# Autodesk Inventor assembly: switchplate-2
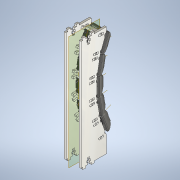
[picture p0: Inventor's stored thumbnail of the model, 180x180]
Saved by Autodesk Inventor 2020.1 (Build 241239000, 239)
## iProperties
Created: 2019-07-06
Part Number: switchplate-2
Document SubType Name: Assembly
Designer: Thibault
Mass: 36.7321 g
Surface Area: 336.688 cm^2
Volume: 13.7102 cm^3
Density: 2.67918 g/cm^3
Author: Thibault
## Documents named in this file (7)
- C:\Users\Thibault Polge\Documents\Habilis\mech\switchplate\switchplate-2.iam
- C:\Users\Thibault Polge\Documents\Habilis\mech\switchplate_support.ipt
- C:\Users\Thibault Polge\Documents\Habilis\mech\mx.iam
- C:\Users\Thibault Polge\Documents\Habilis\mech\extra_switch_support.ipt
- C:\Users\Thibault Polge\Documents\Habilis\mech\mx\DSA-1x1.iam
- C:\Users\Thibault Polge\Documents\Habilis\mech\switchplate.iam
- C:\Users\Thibault Polge\Documents\Habilis\mech\switchplate_support\switchplate-support-02.ipt
## Components (17 placed, 4 different names)
1. switchplate-support:left — Affleurement:1, Affleurement:2, Affleurement:3, Affleurement:5, Affleurement:6, Affleurement:7, Affleurement:8, Affleurement:9, Affleurement:10, Affleurement:11, Affleurement:12, Affleurement:13, Affleurement:14, Affleurement:15, Affleurement:17, Symétrie:1, Affleurement:23, Placage:36, Placage:37, Placage:38, Placage:39, Placage:40, Placage:41, Placage:42, Placage:43, Placage:44, Placage:45, Placage:46, Placage:47, Placage:48, Placage:49, Placage:50
2. Switch:1 [sub-assembly] — Placage:26, Affleurement:22, Placage:35
3. Switch:2 [sub-assembly] — Placage:30, Affleurement:21, Placage:34
4. Switch:3 [sub-assembly] — Placage:27, Affleurement:20, Placage:33
5. Switch:4 [sub-assembly] — Placage:28, Affleurement:19, Placage:32
6. Switch:5 [sub-assembly] — Placage:29, Affleurement:18, Placage:31
7. switchplate-support:right — Affleurement:5, Affleurement:16, Affleurement:17, Symétrie:1, Affleurement:23
8. extra_switch_support:1 — Affleurement:13, Placage:30, Placage:38
9. extra_switch_support:2 — Affleurement:12, Placage:34, Placage:39, Placage:49
10. extra_switch_support:3 — Affleurement:11, Placage:27, Placage:40
11. extra_switch_support:4 — Affleurement:10, Placage:33, Placage:41, Placage:48
12. extra_switch_support:5 — Affleurement:9, Placage:28, Placage:42
13. extra_switch_support:6 — Affleurement:8, Placage:32, Placage:43, Placage:47
14. extra_switch_support:7 — Affleurement:7, Placage:29, Placage:44
15. extra_switch_support:8 — Affleurement:14, Placage:35, Placage:37, Placage:50
16. extra_switch_support:9 — Affleurement:15, Placage:26, Placage:36
17. extra_switch_support:10 — Affleurement:6, Affleurement:16, Placage:31, Placage:45, Placage:46
## Relationships (48: Mate 25, Flush 22, Symmetry 1)
- Affleurement:1 [Flush]: switchplate-support:left
- Affleurement:2 [Flush]: switchplate-support:left
- Affleurement:3 [Flush]: switchplate-support:left
- Affleurement:5 [Flush]: switchplate-support:left ↔ switchplate-support:right
- Affleurement:6 [Flush]: switchplate-support:left ↔ extra_switch_support:10
- Affleurement:7 [Flush]: switchplate-support:left ↔ extra_switch_support:7
- Affleurement:8 [Flush]: switchplate-support:left ↔ extra_switch_support:6
- Affleurement:9 [Flush]: switchplate-support:left ↔ extra_switch_support:5
- Affleurement:10 [Flush]: switchplate-support:left ↔ extra_switch_support:4
- Affleurement:11 [Flush]: switchplate-support:left ↔ extra_switch_support:3
- Affleurement:12 [Flush]: switchplate-support:left ↔ extra_switch_support:2
- Affleurement:13 [Flush]: switchplate-support:left ↔ extra_switch_support:1
- Affleurement:14 [Flush]: switchplate-support:left ↔ extra_switch_support:8
- Affleurement:15 [Flush]: switchplate-support:left ↔ extra_switch_support:9
- Affleurement:16 [Flush]: switchplate-support:right ↔ extra_switch_support:10
- Affleurement:17 [Flush]: switchplate-support:left ↔ switchplate-support:right
- Symétrie:1 [Symmetry]: switchplate-support:left ↔ switchplate-support:right
- Placage:26 [Mate]: Switch:1 ↔ extra_switch_support:9
- Placage:27 [Mate]: Switch:3 ↔ extra_switch_support:3
- Placage:28 [Mate]: Switch:4 ↔ extra_switch_support:5
- Placage:29 [Mate]: Switch:5 ↔ extra_switch_support:7
- Placage:30 [Mate]: Switch:2 ↔ extra_switch_support:1
- Affleurement:18 [Flush]: Switch:5
- Affleurement:19 [Flush]: Switch:4
- Affleurement:20 [Flush]: Switch:3
- Affleurement:21 [Flush]: Switch:2
- Affleurement:22 [Flush]: Switch:1
- Placage:31 [Mate]: Switch:5 ↔ extra_switch_support:10
- Placage:32 [Mate]: Switch:4 ↔ extra_switch_support:6
- Placage:33 [Mate]: Switch:3 ↔ extra_switch_support:4
- Placage:34 [Mate]: Switch:2 ↔ extra_switch_support:2
- Placage:35 [Mate]: Switch:1 ↔ extra_switch_support:8
- Affleurement:23 [Flush]: switchplate-support:left ↔ switchplate-support:right
- Placage:36 [Mate]: switchplate-support:left ↔ extra_switch_support:9
- Placage:37 [Mate]: switchplate-support:left ↔ extra_switch_support:8
- Placage:38 [Mate]: switchplate-support:left ↔ extra_switch_support:1
- Placage:39 [Mate]: switchplate-support:left ↔ extra_switch_support:2
- Placage:40 [Mate]: switchplate-support:left ↔ extra_switch_support:3
- Placage:41 [Mate]: switchplate-support:left ↔ extra_switch_support:4
- Placage:42 [Mate]: switchplate-support:left ↔ extra_switch_support:5
- Placage:43 [Mate]: switchplate-support:left ↔ extra_switch_support:6
- Placage:44 [Mate]: switchplate-support:left ↔ extra_switch_support:7
- Placage:45 [Mate]: switchplate-support:left ↔ extra_switch_support:10
- Placage:46 [Mate]: switchplate-support:left ↔ extra_switch_support:10
- Placage:47 [Mate]: switchplate-support:left ↔ extra_switch_support:6
- Placage:48 [Mate]: switchplate-support:left ↔ extra_switch_support:4
- Placage:49 [Mate]: switchplate-support:left ↔ extra_switch_support:2
- Placage:50 [Mate]: switchplate-support:left ↔ extra_switch_support:8
